# Autodesk Inventor assembly: Piso e tampa dos motores
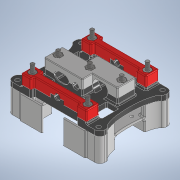
[picture p0: Inventor's stored thumbnail of the model, 180x180]
Saved by Autodesk Inventor 2021 (Build 250183000, 183)
## iProperties
Created: 2022-02-01
Part Number: Piso e tampa dos motores
Document SubType Name: Assembly
Designer: Matheus
Author: Matheus
## Documents named in this file (7)
- D:\Projetos\Red Dragons 22\Piso e tampa dos motores.iam
- D:\Projetos\Red Dragons 22\Piso dos motores.ipt
- D:\Projetos\Red Dragons 22\Tampa motores.ipt
- D:\Projetos\Red Dragons 22\Porca - M3 x 0,5.ipt
- D:\Projetos\Red Dragons 22\Parafuso - M3x0,5 x 20.ipt
- D:\Projetos\Red Dragons 22\Mancal superior.ipt
- D:\Projetos\Red Dragons 22\Suporte Ball Caster Max.ipt
## Components (20 placed, 6 different names)
1. Piso dos motores:1 — Mate:1, Mate:2, Mate:3, Mate:10, Flush:1, Mate:11, Flush:2, Mate:12, Flush:3, Mate:13, Mate:14, Mate:15, Mate:16, Mate:17, Mate:18, Flush:4, Mate:20, Flush:5, Mate:21, Flush:6, Mate:22, Flush:7, Mate:31, Mate:32, Mate:33, Mate:34, Mate:35, Mate:36
2. Tampa motores:1 — Mate:1, Mate:2, Mate:3, Mate:4, Mate:5, Angle:1, Mate:6, Mate:7, Angle:2, Mate:8, Mate:9, Angle:3
3. Porca - M3 x 0,5:1 — Mate:4, Mate:5, Angle:1
4. Porca - M3 x 0,5:2 — Mate:8, Mate:9, Angle:3
5. Porca - M3 x 0,5:3 — Mate:6, Mate:7, Angle:2
6. Parafuso - M3x0,5 x 20:1 — Mate:11, Flush:2
7. Parafuso - M3x0,5 x 20:2 — Mate:10, Flush:1
8. Parafuso - M3x0,5 x 20:3 — Mate:12, Flush:3
9. Mancal superior:1 — Mate:16, Mate:17, Mate:18, Mate:28, Angle:6, Mate:30, Angle:7
10. Mancal superior:2 — Mate:13, Mate:14, Mate:15, Mate:19, Mate:24, Angle:4, Mate:26, Angle:5
11. Parafuso - M3x0,5 x 20:4 — Mate:19, Flush:4, Mate:23
12. Parafuso - M3x0,5 x 20:5 — Mate:20, Flush:5, Mate:25
13. Parafuso - M3x0,5 x 20:6 — Mate:22, Flush:7, Mate:27
14. Parafuso - M3x0,5 x 20:7 — Mate:21, Flush:6, Mate:29
15. Porca - M3 x 0,5:4 — Mate:23, Mate:24, Angle:4
16. Porca - M3 x 0,5:5 — Mate:25, Mate:26, Angle:5
17. Porca - M3 x 0,5:6 — Mate:29, Mate:30, Angle:7
18. Porca - M3 x 0,5:7 — Mate:27, Mate:28, Angle:6
19. Suporte Ball Caster Max:1 — Mate:31, Mate:32, Mate:33
20. Suporte Ball Caster Max:2 — Mate:34, Mate:35, Mate:36
## Relationships (50: Mate 36, Angle 7, Flush 7)
- Mate:1: Piso dos motores:1 ↔ Tampa motores:1
- Mate:2: Piso dos motores:1 ↔ Tampa motores:1
- Mate:3: Piso dos motores:1 ↔ Tampa motores:1
- Mate:4: Tampa motores:1 ↔ Porca - M3 x 0,5:1
- Mate:5: Tampa motores:1 ↔ Porca - M3 x 0,5:1
- Angle:1 (0 deg): Tampa motores:1 ↔ Porca - M3 x 0,5:1
- Mate:6: Tampa motores:1 ↔ Porca - M3 x 0,5:3
- Mate:7: Tampa motores:1 ↔ Porca - M3 x 0,5:3
- Angle:2 (0 deg): Tampa motores:1 ↔ Porca - M3 x 0,5:3
- Mate:8: Tampa motores:1 ↔ Porca - M3 x 0,5:2
- Mate:9: Tampa motores:1 ↔ Porca - M3 x 0,5:2
- Angle:3 (0 deg): Tampa motores:1 ↔ Porca - M3 x 0,5:2
- Mate:10: Piso dos motores:1 ↔ Parafuso - M3x0,5 x 20:2
- Flush:1: Piso dos motores:1 ↔ Parafuso - M3x0,5 x 20:2
- Mate:11: Piso dos motores:1 ↔ Parafuso - M3x0,5 x 20:1
- Flush:2: Piso dos motores:1 ↔ Parafuso - M3x0,5 x 20:1
- Mate:12: Piso dos motores:1 ↔ Parafuso - M3x0,5 x 20:3
- Flush:3: Piso dos motores:1 ↔ Parafuso - M3x0,5 x 20:3
- Mate:13: Piso dos motores:1 ↔ Mancal superior:2
- Mate:14: Piso dos motores:1 ↔ Mancal superior:2
- Mate:15: Piso dos motores:1 ↔ Mancal superior:2
- Mate:16: Piso dos motores:1 ↔ Mancal superior:1
- Mate:17: Piso dos motores:1 ↔ Mancal superior:1
- Mate:18: Piso dos motores:1 ↔ Mancal superior:1
- Mate:19: Mancal superior:2 ↔ Parafuso - M3x0,5 x 20:4
- Flush:4: Piso dos motores:1 ↔ Parafuso - M3x0,5 x 20:4
- Mate:20: Piso dos motores:1 ↔ Parafuso - M3x0,5 x 20:5
- Flush:5: Piso dos motores:1 ↔ Parafuso - M3x0,5 x 20:5
- Mate:21: Piso dos motores:1 ↔ Parafuso - M3x0,5 x 20:7
- Flush:6: Piso dos motores:1 ↔ Parafuso - M3x0,5 x 20:7
- Mate:22: Piso dos motores:1 ↔ Parafuso - M3x0,5 x 20:6
- Flush:7: Piso dos motores:1 ↔ Parafuso - M3x0,5 x 20:6
- Mate:23: Parafuso - M3x0,5 x 20:4 ↔ Porca - M3 x 0,5:4
- Mate:24: Mancal superior:2 ↔ Porca - M3 x 0,5:4
- Angle:4 (0 deg): Mancal superior:2 ↔ Porca - M3 x 0,5:4
- Mate:25: Parafuso - M3x0,5 x 20:5 ↔ Porca - M3 x 0,5:5
- Mate:26: Mancal superior:2 ↔ Porca - M3 x 0,5:5
- Angle:5 (0 deg): Mancal superior:2 ↔ Porca - M3 x 0,5:5
- Mate:27: Parafuso - M3x0,5 x 20:6 ↔ Porca - M3 x 0,5:7
- Mate:28: Mancal superior:1 ↔ Porca - M3 x 0,5:7
- Angle:6 (0 deg): Mancal superior:1 ↔ Porca - M3 x 0,5:7
- Mate:29: Parafuso - M3x0,5 x 20:7 ↔ Porca - M3 x 0,5:6
- Mate:30: Mancal superior:1 ↔ Porca - M3 x 0,5:6
- Angle:7 (0 deg): Mancal superior:1 ↔ Porca - M3 x 0,5:6
- Mate:31: Piso dos motores:1 ↔ Suporte Ball Caster Max:1
- Mate:32: Piso dos motores:1 ↔ Suporte Ball Caster Max:1
- Mate:33: Piso dos motores:1 ↔ Suporte Ball Caster Max:1
- Mate:34: Piso dos motores:1 ↔ Suporte Ball Caster Max:2
- Mate:35: Piso dos motores:1 ↔ Suporte Ball Caster Max:2
- Mate:36: Piso dos motores:1 ↔ Suporte Ball Caster Max:2
